# Autodesk Inventor assembly: Shadow_Game
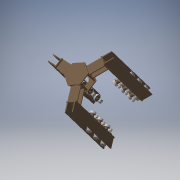
[picture p0: Inventor's stored thumbnail of the model, 180x180]
Saved by Autodesk Inventor 2016 (Build 200138000, 138)
## iProperties
Created: 2016-01-06
Part Number: Shadow_Game
Document SubType Name: Assembly
Designer: m2memari
Author: m2memari
## Documents named in this file (8)
- C:\MoDonGD\Jane\ShadowGame\ShadowGame\Shadow_Game.iam
- C:\MoDonGD\Jane\ShadowGame\ShadowGame\Motor_Bar.iam
- C:\MoDonGD\Jane\ShadowGame\ShadowGame\SPG30_Motor.ipt
- C:\MoDonGD\Jane\ShadowGame\ShadowGame\MotorCoupling.iam
- C:\MoDonGD\Jane\ShadowGame\ShadowGame\Bearing_Silicone.ipt
- C:\MoDonGD\Jane\ShadowGame\ShadowGame\IBeam.iam
- C:\MoDonGD\Jane\ShadowGame\ShadowGame\LightDiskBottom.ipt
- C:\MoDonGD\Jane\ShadowGame\ShadowGame\LightDiskTop.ipt
## Components (44 placed, 7 different names)
1. Motor_Bar:3 [sub-assembly] — Mate:64, Mate:65, Mate:66
2. SPG30_Motor:7
3. MotorCoupling:7 [sub-assembly]
4. MotorCoupling:8 [sub-assembly]
5. SPG30_Motor:8
6. SPG30_Motor:9
7. MotorCoupling:9 [sub-assembly]
8. Bearing_Silicone:13
9. Bearing_Silicone:14
10. Bearing_Silicone:15
11. Bearing_Silicone:16
12. Bearing_Silicone:17
13. Bearing_Silicone:18
14. IBeam:1 [sub-assembly] — Mate:64, Mate:65, Mate:66, Mate:139, Mate:140, Mate:141
15. Motor_Bar:4 [sub-assembly]
16. SPG30_Motor:10
17. MotorCoupling:10 [sub-assembly]
18. MotorCoupling:11 [sub-assembly]
19. SPG30_Motor:11
20. SPG30_Motor:12
21. MotorCoupling:12 [sub-assembly]
22. Bearing_Silicone:19
23. Bearing_Silicone:20
24. Bearing_Silicone:21
25. Bearing_Silicone:22
26. Bearing_Silicone:23
27. Bearing_Silicone:24
28. IBeam:2 [sub-assembly] — Mate:142, Mate:143, Mate:144, Mate:148, Mate:149, Mate:150
29. Motor_Bar:6 [sub-assembly]
30. SPG30_Motor:16
31. MotorCoupling:16 [sub-assembly]
32. MotorCoupling:17 [sub-assembly]
33. SPG30_Motor:17
34. SPG30_Motor:18
35. MotorCoupling:18 [sub-assembly]
36. Bearing_Silicone:31
37. Bearing_Silicone:32
38. Bearing_Silicone:33
39. Bearing_Silicone:34
40. Bearing_Silicone:35
41. Bearing_Silicone:36
42. IBeam:4 [sub-assembly] — Mate:145, Mate:146, Mate:147
43. LightDiskBottom:1 — Mate:148, Mate:149, Mate:150
44. LightDiskTop:1 — Mate:139, Mate:140, Mate:141, Mate:142, Mate:143, Mate:144, Mate:145, Mate:146, Mate:147
## Relationships (99: Mate 84, Flush 9, Insert 3, Tangent 3)
- [Insert]: Motor_Bar:3 ↔ SPG30_Motor:7
- [Tangent]: Motor_Bar:3 ↔ SPG30_Motor:7
- [Mate]: SPG30_Motor:7 ↔ MotorCoupling:7
- [Flush]: Motor_Bar:3 ↔ MotorCoupling:7
- [Mate]: Motor_Bar:3 ↔ SPG30_Motor:9
- [Mate]: Motor_Bar:3 ↔ SPG30_Motor:8
- [Mate]: Motor_Bar:3 ↔ SPG30_Motor:9
- [Mate]: Motor_Bar:3 ↔ SPG30_Motor:8
- [Mate]: Motor_Bar:3 ↔ SPG30_Motor:9
- [Mate]: Motor_Bar:3 ↔ SPG30_Motor:8
- [Mate]: SPG30_Motor:9 ↔ MotorCoupling:9
- [Mate]: MotorCoupling:8 ↔ SPG30_Motor:8
- [Flush]: Motor_Bar:3 ↔ MotorCoupling:9
- [Flush]: Motor_Bar:3 ↔ MotorCoupling:8
- [Mate]: Motor_Bar:3 ↔ Bearing_Silicone:13
- [Mate]: Motor_Bar:3 ↔ Bearing_Silicone:13
- [Mate]: Motor_Bar:3 ↔ Bearing_Silicone:14
- [Mate]: Motor_Bar:3 ↔ Bearing_Silicone:15
- [Mate]: Motor_Bar:3 ↔ Bearing_Silicone:16
- [Mate]: Motor_Bar:3 ↔ Bearing_Silicone:17
- [Mate]: Motor_Bar:3 ↔ Bearing_Silicone:18
- [Mate]: Motor_Bar:3 ↔ Bearing_Silicone:14
- [Mate]: Motor_Bar:3 ↔ Bearing_Silicone:15
- [Mate]: Motor_Bar:3 ↔ Bearing_Silicone:16
- [Mate]: Motor_Bar:3 ↔ Bearing_Silicone:17
- [Mate]: Motor_Bar:3 ↔ Bearing_Silicone:18
- Mate:64: Motor_Bar:3 ↔ IBeam:1
- Mate:65: Motor_Bar:3 ↔ IBeam:1
- Mate:66: Motor_Bar:3 ↔ IBeam:1
- [Insert]: Motor_Bar:4 ↔ SPG30_Motor:10
- [Tangent]: Motor_Bar:4 ↔ SPG30_Motor:10
- [Mate]: SPG30_Motor:10 ↔ MotorCoupling:10
- [Flush]: Motor_Bar:4 ↔ MotorCoupling:10
- [Mate]: Motor_Bar:4 ↔ SPG30_Motor:12
- [Mate]: Motor_Bar:4 ↔ SPG30_Motor:11
- [Mate]: Motor_Bar:4 ↔ SPG30_Motor:12
- [Mate]: Motor_Bar:4 ↔ SPG30_Motor:11
- [Mate]: Motor_Bar:4 ↔ SPG30_Motor:12
- [Mate]: Motor_Bar:4 ↔ SPG30_Motor:11
- [Mate]: SPG30_Motor:12 ↔ MotorCoupling:12
- [Mate]: MotorCoupling:11 ↔ SPG30_Motor:11
- [Flush]: Motor_Bar:4 ↔ MotorCoupling:12
- [Flush]: Motor_Bar:4 ↔ MotorCoupling:11
- [Mate]: Motor_Bar:4 ↔ Bearing_Silicone:19
- [Mate]: Motor_Bar:4 ↔ Bearing_Silicone:19
- [Mate]: Motor_Bar:4 ↔ Bearing_Silicone:20
- [Mate]: Motor_Bar:4 ↔ Bearing_Silicone:21
- [Mate]: Motor_Bar:4 ↔ Bearing_Silicone:22
- [Mate]: Motor_Bar:4 ↔ Bearing_Silicone:23
- [Mate]: Motor_Bar:4 ↔ Bearing_Silicone:24
- [Mate]: Motor_Bar:4 ↔ Bearing_Silicone:20
- [Mate]: Motor_Bar:4 ↔ Bearing_Silicone:21
- [Mate]: Motor_Bar:4 ↔ Bearing_Silicone:22
- [Mate]: Motor_Bar:4 ↔ Bearing_Silicone:23
- [Mate]: Motor_Bar:4 ↔ Bearing_Silicone:24
- [Mate]: Motor_Bar:4 ↔ IBeam:2
- [Mate]: Motor_Bar:4 ↔ IBeam:2
- [Mate]: Motor_Bar:4 ↔ IBeam:2
- [Insert]: Motor_Bar:6 ↔ SPG30_Motor:16
- [Tangent]: Motor_Bar:6 ↔ SPG30_Motor:16
- [Mate]: SPG30_Motor:16 ↔ MotorCoupling:16
- [Flush]: Motor_Bar:6 ↔ MotorCoupling:16
- [Mate]: Motor_Bar:6 ↔ SPG30_Motor:18
- [Mate]: Motor_Bar:6 ↔ SPG30_Motor:17
- [Mate]: Motor_Bar:6 ↔ SPG30_Motor:18
- [Mate]: Motor_Bar:6 ↔ SPG30_Motor:17
- [Mate]: Motor_Bar:6 ↔ SPG30_Motor:18
- [Mate]: Motor_Bar:6 ↔ SPG30_Motor:17
- [Mate]: SPG30_Motor:18 ↔ MotorCoupling:18
- [Mate]: MotorCoupling:17 ↔ SPG30_Motor:17
- [Flush]: Motor_Bar:6 ↔ MotorCoupling:18
- [Flush]: Motor_Bar:6 ↔ MotorCoupling:17
- [Mate]: Motor_Bar:6 ↔ Bearing_Silicone:31
- [Mate]: Motor_Bar:6 ↔ Bearing_Silicone:31
- [Mate]: Motor_Bar:6 ↔ Bearing_Silicone:32
- [Mate]: Motor_Bar:6 ↔ Bearing_Silicone:33
- [Mate]: Motor_Bar:6 ↔ Bearing_Silicone:34
- [Mate]: Motor_Bar:6 ↔ Bearing_Silicone:35
- [Mate]: Motor_Bar:6 ↔ Bearing_Silicone:36
- [Mate]: Motor_Bar:6 ↔ Bearing_Silicone:32
- [Mate]: Motor_Bar:6 ↔ Bearing_Silicone:33
- [Mate]: Motor_Bar:6 ↔ Bearing_Silicone:34
- [Mate]: Motor_Bar:6 ↔ Bearing_Silicone:35
- [Mate]: Motor_Bar:6 ↔ Bearing_Silicone:36
- [Mate]: Motor_Bar:6 ↔ IBeam:4
- [Mate]: Motor_Bar:6 ↔ IBeam:4
- [Mate]: Motor_Bar:6 ↔ IBeam:4
- Mate:139: IBeam:1 ↔ LightDiskTop:1
- Mate:140: IBeam:1 ↔ LightDiskTop:1
- Mate:141: IBeam:1 ↔ LightDiskTop:1
- Mate:142: IBeam:2 ↔ LightDiskTop:1
- Mate:143: IBeam:2 ↔ LightDiskTop:1
- Mate:144: IBeam:2 ↔ LightDiskTop:1
- Mate:145: IBeam:4 ↔ LightDiskTop:1
- Mate:146: IBeam:4 ↔ LightDiskTop:1
- Mate:147: IBeam:4 ↔ LightDiskTop:1
- Mate:148: IBeam:2 ↔ LightDiskBottom:1
- Mate:149: IBeam:2 ↔ LightDiskBottom:1
- Mate:150: IBeam:2 ↔ LightDiskBottom:1
## Named parameters: d58_d20 = 0 mm, d59_d21 = 0 mm, d60_d22 = 0 mm, d61_d23 = 0 mm, d62_d24 = 0 mm, d63_d25 = 0 mm, d64_d26 = 0 mm, d65_d27 = 0 mm, d66_d28 = 0 mm, d67_d29 = 0 mm, d68_d30 = 0 mm, d69_d31 = 0 mm, d70_d15 = 0 mm, d71_d4 = 0 mm, d72_d5 = 0 mm, d73_d6 = 0 mm, d74_d7 = 0 mm, d75_d8 = 0 mm, d76_d9 = 0 mm, d77_d10 = 0 mm, d78_d11 = 0 mm, d79_d12 = 0 mm, d80_d13 = 0 mm, d81_d14 = 0 mm, d82_d0 = 0 mm, d83_d1 = 0 mm, d87_d84 = 0 mm, d88_d85 = 0 mm, d89_d86 = 0 mm, d90_d58_d20 = 0 mm, d91_d59_d21 = 0 mm, d92_d60_d22 = 0 mm, d93_d61_d23 = 0 mm, d94_d62_d24 = 0 mm, d95_d63_d25 = 0 mm, d96_d64_d26 = 0 mm, d97_d65_d27 = 0 mm, d98_d66_d28 = 0 mm, d99_d67_d29 = 0 mm, d100_d68_d30 = 0 mm, d101_d69_d31 = 0 mm, d102_d70_d15 = 0 mm, d103_d71_d4 = 0 mm, d104_d72_d5 = 0 mm, d105_d73_d6 = 0 mm, d106_d74_d7 = 0 mm, d107_d75_d8 = 0 mm, d108_d76_d9 = 0 mm, d109_d77_d10 = 0 mm, d110_d78_d11 = 0 mm, d111_d79_d12 = 0 mm, d112_d80_d13 = 0 mm, d113_d81_d14 = 0 mm, d114_d82_d0 = 0 mm, d115_d83_d1 = 0 mm, d145_d84 = 0 mm, d146_d85 = 0 mm, d147_d86 = 0 mm, d148_d58_d20 = 0 mm, d149_d59_d21 = 0 mm, d150_d60_d22 = 0 mm, d151_d61_d23 = 0 mm, d152_d62_d24 = 0 mm, d153_d63_d25 = 0 mm, d154_d64_d26 = 0 mm, d155_d65_d27 = 0 mm, d156_d66_d28 = 0 mm, d157_d67_d29 = 0 mm, d158_d68_d30 = 0 mm, d159_d69_d31 = 0 mm, d160_d70_d15 = 0 mm, d161_d71_d4 = 0 mm, d162_d72_d5 = 0 mm, d163_d73_d6 = 0 mm, d164_d74_d7 = 0 mm, d165_d75_d8 = 0 mm, d166_d76_d9 = 0 mm, d167_d77_d10 = 0 mm, d168_d78_d11 = 0 mm, d169_d79_d12 = 0 mm, d170_d80_d13 = 0 mm, d171_d81_d14 = 0 mm, d172_d82_d0 = 0 mm, d173_d83_d1 = 0 mm
